# Autodesk Inventor assembly: bayonet
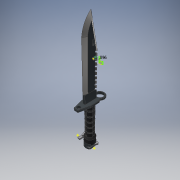
[picture p0: Inventor's stored thumbnail of the model, 180x180]
Saved by Autodesk Inventor 2018 (Build 220112000, 112)
## iProperties
Created: 2020-12-01
Part Number: bayonet
Material: Všeobecné
Document SubType Name: Assembly
Designer: Jozko Mrkvicka
Author: Jozko Mrkvicka
## Documents named in this file (10)
- F:\Workspace\05_Projekty\Bayonet\bayonet.iam
- F:\Workspace\05_Projekty\Bayonet\blade.ipt
- F:\Workspace\05_Projekty\Bayonet\crossguard.ipt
- F:\Workspace\05_Projekty\Bayonet\handle.ipt
- F:\Workspace\05_Projekty\Bayonet\attachment.ipt
- F:\Workspace\05_Projekty\Bayonet\pin.ipt
- F:\Workspace\05_Projekty\Bayonet\nut.ipt
- F:\Workspace\05_Projekty\Common\Library_Inventor\Bolt-M3x20.ipt
- F:\Workspace\05_Projekty\Common\Library_Inventor\Nut-M3.ipt
- F:\Workspace\05_Projekty\Common\Library_Inventor\LED-5mm-Green.ipt
## Components (12 placed, 9 different names)
1. blade:1 — Proti sobě:8, Proti sobě:9, Proti sobě:10, Proti sobě:11, Proti sobě:12, Vložit:5
2. crossguard:1 — Proti sobě:8, Proti sobě:9, Proti sobě:10, Proti sobě:13
3. handle:1 — Proti sobě:11, Proti sobě:12, Proti sobě:13, Proti sobě:14
4. attachment:1 — Vložit:1, Vložit:2, Proti sobě:14, Vložit:4, Vložit:6, Vložit:7, Vložit:8, Proti sobě:15, Vložit:9, Proti sobě:16, Vložit:10
5. pin:1 — Rotace:1, Vložit:1, Vložit:10
6. pin:2 — Rotace:1, Vložit:2
7. nut:1 — Vložit:4, Vložit:5
8. Bolt-M3x20:1 — Vložit:6
9. Bolt-M3x20:2 — Vložit:7
10. Nut-M3:1 — Vložit:8, Proti sobě:15
11. Nut-M3:2 — Vložit:9, Proti sobě:16
12. LED-5mm-Green:1
## Relationships (19: Insert 9, Mate 9, RelateRotation 1)
- Rotace:1 [RelateRotation] (1 ul): pin:1 ↔ pin:2
- Vložit:1 [Insert]: attachment:1 ↔ pin:1
- Vložit:2 [Insert]: attachment:1 ↔ pin:2
- Proti sobě:8 [Mate]: blade:1 ↔ crossguard:1
- Proti sobě:9 [Mate]: blade:1 ↔ crossguard:1
- Proti sobě:10 [Mate]: blade:1 ↔ crossguard:1
- Proti sobě:11 [Mate]: blade:1 ↔ handle:1
- Proti sobě:12 [Mate]: blade:1 ↔ handle:1
- Proti sobě:13 [Mate]: crossguard:1 ↔ handle:1
- Proti sobě:14 [Mate]: handle:1 ↔ attachment:1
- Vložit:4 [Insert]: attachment:1 ↔ nut:1
- Vložit:5 [Insert]: blade:1 ↔ nut:1
- Vložit:6 [Insert]: attachment:1 ↔ Bolt-M3x20:1
- Vložit:7 [Insert]: attachment:1 ↔ Bolt-M3x20:2
- Vložit:8 [Insert]: attachment:1 ↔ Nut-M3:1
- Proti sobě:15 [Mate]: attachment:1 ↔ Nut-M3:1
- Vložit:9 [Insert]: attachment:1 ↔ Nut-M3:2
- Proti sobě:16 [Mate]: attachment:1 ↔ Nut-M3:2
- Vložit:10 [Insert]: attachment:1 ↔ pin:1
